# Autodesk Inventor assembly: GateLEDBox
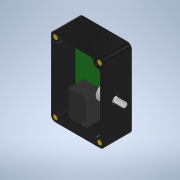
[picture p0: Inventor's stored thumbnail of the model, 180x180]
Saved by Autodesk Inventor 2021 (Build 250183000, 183)
## iProperties
Created: 2021-02-15
Part Number: GateLEDBox
Document SubType Name: Assembly
Designer: James
Author: James
## Documents named in this file (7)
- C:\Users\james\Dev\homeprojects\Electronics\XC-0001-Gate_LEDs Rev 2\3D model\GateLEDBox.iam
- C:\Users\james\Dev\homeprojects\Electronics\3D Model\PinfoxBox.ipt
- C:\Users\james\Dev\homeprojects\Electronics\3D Model\ThreadedInsertM4\M4 threaded insert.ipt
- C:\Users\james\Dev\homeprojects\Electronics\3D Model\ThreadedInsertM4\M4 threaded insert_MIR.ipt
- C:\Users\james\Dev\homeprojects\Electronics\3D Model\ThreadedInsertM4\M4 threaded insert_MIR1.ipt
- C:\Users\james\Dev\homeprojects\Electronics\3D Model\ThreadedInsertM4\M4 threaded insert_MIR_MIR.ipt
- C:\Users\james\Dev\homeprojects\Electronics\XC-0001-Gate_LEDs Rev 2\3D export\XC-0001-Gate_LEDs.iam
## Components (6 placed, 6 different names)
1. PinfoxBox:1 — Flush:1, Flush:2, Flush:3, Insert:1, Mate:1, Mate:2
2. M4 threaded insert:1 — Insert:1
3. M4 threaded insert_MIR:1
4. M4 threaded insert_MIR1:1
5. M4 threaded insert_MIR_MIR:1
6. XC-0001-Gate_LEDs:1 [sub-assembly] — Mate:1, Mate:2
## Relationships (6: Flush 3, Mate 2, Insert 1)
- Flush:1: PinfoxBox:1
- Flush:2: PinfoxBox:1
- Flush:3: PinfoxBox:1
- Insert:1: PinfoxBox:1 ↔ M4 threaded insert:1
- Mate:1: PinfoxBox:1 ↔ XC-0001-Gate_LEDs:1
- Mate:2: PinfoxBox:1 ↔ XC-0001-Gate_LEDs:1
